# Autodesk Inventor assembly: NikkonTubelensBridge
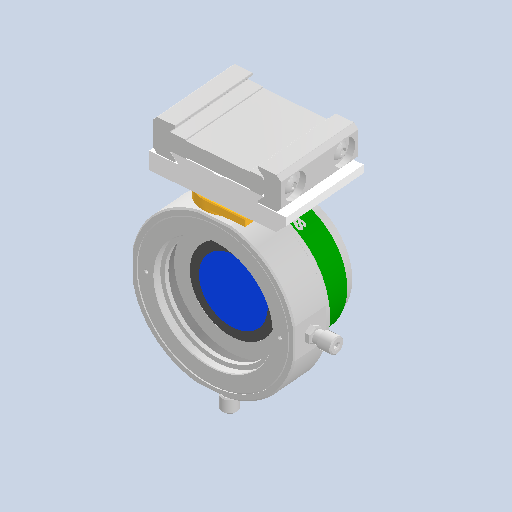
[picture p0: Inventor's stored thumbnail of the model, 512x512]
Saved by Autodesk Inventor 2026.1 (Build 301233000, 233)
## iProperties
Created: 2019-08-20
Part Number: NikkonTubelensBridge
Document SubType Name: Assembly
Designer: Julian
Author: Julian
## Documents named in this file (5)
- C:\Users\user\Desktop\setup_inventor_2025\LightPath\lens\NikkonTubelensBridge.iam
- C:\Users\user\Desktop\setup_inventor_2025\LightPath\lens\XT66C2-Step_rail mount.ipt
- C:\Users\user\Desktop\setup_inventor_2025\LightPath\lens\NikkonTubelensAssembly.iam
- C:\Users\user\Desktop\setup_inventor_2025\LightPath\lens\XT66D2-40-Step_post_mount_lens_adj.ipt
- C:\Users\user\Desktop\setup_inventor_2025\LightPath\lens\M-PS-KF_miroor_flip.ipt
## Components (4 placed, 4 different names)
1. XT66C2-Step_rail mount:1 — Passend:7, Passend:8, Fluchtend:1
2. NikkonTubelensAssembly:1 [sub-assembly] — Winkel:1, Passend:11, Passend:12
3. XT66D2-40-Step_post_mount_lens_adj:1 — Passend:7, Passend:8, Fluchtend:1, Winkel:1, Passend:9, Passend:10, Winkel:2
4. M-PS-KF_miroor_flip:1 — Passend:9, Passend:10, Passend:11, Passend:12, Winkel:2
## Relationships (9: Mate 6, Angle 2, Flush 1)
- Passend:7 [Mate]: XT66C2-Step_rail mount:1 ↔ XT66D2-40-Step_post_mount_lens_adj:1
- Passend:8 [Mate]: XT66C2-Step_rail mount:1 ↔ XT66D2-40-Step_post_mount_lens_adj:1
- Fluchtend:1 [Flush]: XT66C2-Step_rail mount:1 ↔ XT66D2-40-Step_post_mount_lens_adj:1
- Winkel:1 [Angle] (0 deg): NikkonTubelensAssembly:1 ↔ XT66D2-40-Step_post_mount_lens_adj:1
- Passend:9 [Mate]: XT66D2-40-Step_post_mount_lens_adj:1 ↔ M-PS-KF_miroor_flip:1
- Passend:10 [Mate]: XT66D2-40-Step_post_mount_lens_adj:1 ↔ M-PS-KF_miroor_flip:1
- Passend:11 [Mate]: NikkonTubelensAssembly:1 ↔ M-PS-KF_miroor_flip:1
- Passend:12 [Mate]: NikkonTubelensAssembly:1 ↔ M-PS-KF_miroor_flip:1
- Winkel:2 [Angle] (0 deg): XT66D2-40-Step_post_mount_lens_adj:1 ↔ M-PS-KF_miroor_flip:1
